# Autodesk Inventor assembly: СборкаЩитков
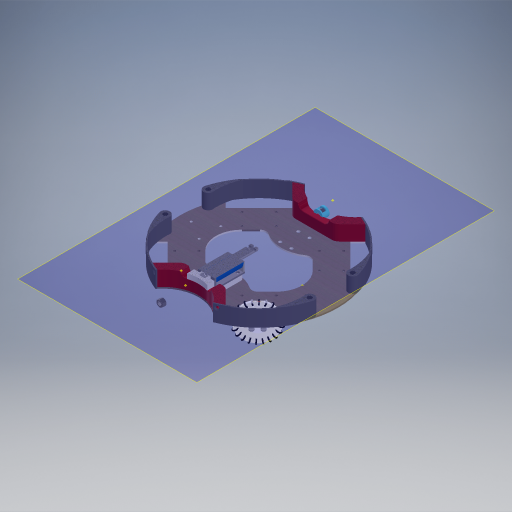
[picture p0: Inventor's stored thumbnail of the model, 512x512]
Saved by Autodesk Inventor 2023 (Build 270158000, 158)
## iProperties
Created: 2025-03-26
Part Number: СборкаЩитков
Document SubType Name: Assembly
Designer: Ivan
Author: Ivan
## Documents named in this file (14)
- C:\!projects\dash_localDirectory\DASH_\Dash-V1\СборкаЩитков.iam
- C:\!projects\dash_localDirectory\DASH_\Dash-V1\step\m3_bolt\СтойкаКруглая.iam
- C:\!projects\dash_localDirectory\DASH_\Dash-V1\floor_v3.ipt
- C:\!projects\dash_localDirectory\DASH_\Dash-V1\contour_v2.ipt
- C:\!projects\dash_localDirectory\DASH_\Dash-V1\protect_v2.2.ipt
- C:\!projects\dash_localDirectory\DASH_\Dash-V1\protect_v2.2_dash.ipt
- C:\!projects\dash_localDirectory\DASH_\Dash-V1\catch_v2.ipt
- C:\!projects\dash_localDirectory\DASH_\Dash-V1\Solenoid\kicker.ipt
- C:\Users\Ivan\Documents\Inventor\Content Center Files\R2023\ru-RU\ANSI B18.2.4.2M\ANSI B18.2.4.2M - M5x0,8 - 8.ipt
- C:\!projects\dash_localDirectory\DASH_\Dash-V1\Solenoid\kicker_MIR.ipt
- C:\!projects\dash_localDirectory\DASH_\Dash-V1\wheel\Wheel.iam
- C:\!projects\DASH-\3D\Dash-V1\Solenoid\Подставка под солноид.ipt
- C:\!projects\DASH-\3D\Dash-V1\Solenoid\Solenoid.iam
- C:\!projects\DASH-\3D\Dash-V1\Solenoid\kicker1.1.ipt
## Components (20 placed, 12 different names)
1. СтойкаКруглая:1 [sub-assembly] — Вставка:19, Вставка:21
2. СтойкаКруглая:2 [sub-assembly] — Вставка:17, Вставка:23
3. СтойкаКруглая:3 [sub-assembly] — Вставка:16, Вставка:22
4. СтойкаКруглая:4 [sub-assembly] — Вставка:18, Вставка:20
5. floor_v3:1 — Вставка:11, Вставка:12, Вставка:13, Касательность:1, Касательность:2, Касательность:3, Касательность:4, Совмещение:6, Совмещение:9, Совмещение:10, Совмещение:11, Вставка:26
6. contour:1 — Вставка:14, Вставка:15, Вставка:16, Вставка:17, Вставка:18, Вставка:19, Угол:2, Совмещение:4, Совмещение:5, Совмещение:7, Совмещение:8
7. protect_v2:1 — Вставка:22, Касательность:1
8. protect_v2:2 — Вставка:20, Касательность:2
9. protect_v2:3 — Вставка:21, Касательность:4
10. protect_v2:4 — Касательность:3, Вставка:23, Совмещение:1, Совмещение:2
11. catch_v2:1 — Вставка:12, Вставка:13, Вставка:15, Совмещение:3
12. catch_v2:2 — Вставка:11, Вставка:14, Совмещение:1, Совмещение:2, Совмещение:13, Заподлицо:2, Совмещение:16
13. kicker:1 — Совмещение:3, Вставка:24, Угол:1, Угол:2
14. ANSI B18.2.4.2M M5x0,8:1 — Вставка:24, Угол:1
15. kicker_MIR:1 — Угол:3, Вставка:25
16. ANSI B18.2.4.2M M5x0,8:2 — Угол:3, Вставка:25
17. Wheel:1 [sub-assembly] — Совмещение:10
18. Подставка под солноид:1 — Совмещение:11, Вставка:26, Совмещение:12, Угол:4, Вставка:27
19. Solenoid:1 [sub-assembly] — Совмещение:12, Угол:4, Вставка:27, Заподлицо:1
20. kicker1.1:1 — Заподлицо:1, Совмещение:13, Заподлицо:2, Совмещение:14, Совмещение:15
## Relationships (43: Insert 17, Mate 16, Tangent 4, Angle 4, Flush 2)
- Вставка:11 [Insert]: floor_v3:1 ↔ catch_v2:2
- Вставка:12 [Insert]: floor_v3:1 ↔ catch_v2:1
- Вставка:13 [Insert]: floor_v3:1 ↔ catch_v2:1
- Вставка:14 [Insert]: contour:1 ↔ catch_v2:2
- Вставка:15 [Insert]: contour:1 ↔ catch_v2:1
- Вставка:16 [Insert]: СтойкаКруглая:3 ↔ contour:1
- Вставка:17 [Insert]: СтойкаКруглая:2 ↔ contour:1
- Вставка:18 [Insert]: СтойкаКруглая:4 ↔ contour:1
- Вставка:19 [Insert]: СтойкаКруглая:1 ↔ contour:1
- Вставка:20 [Insert]: СтойкаКруглая:4 ↔ protect_v2:2
- Вставка:21 [Insert]: СтойкаКруглая:1 ↔ protect_v2:3
- Вставка:22 [Insert]: СтойкаКруглая:3 ↔ protect_v2:1
- Касательность:1 [Tangent]: floor_v3:1 ↔ protect_v2:1
- Касательность:2 [Tangent]: floor_v3:1 ↔ protect_v2:2
- Касательность:3 [Tangent]: floor_v3:1 ↔ protect_v2:4
- Вставка:23 [Insert]: СтойкаКруглая:2 ↔ protect_v2:4
- Касательность:4 [Tangent]: floor_v3:1 ↔ protect_v2:3
- Совмещение:1 [Mate]: protect_v2:4 ↔ catch_v2:2
- Совмещение:2 [Mate]: protect_v2:4 ↔ catch_v2:2
- Совмещение:3 [Mate]: catch_v2:1 ↔ kicker:1
- Вставка:24 [Insert]: kicker:1 ↔ ANSI B18.2.4.2M M5x0,8:1
- Угол:1 [Angle] (0 deg): kicker:1 ↔ ANSI B18.2.4.2M M5x0,8:1
- Угол:2 [Angle] (90 deg): contour:1 ↔ kicker:1
- Совмещение:4 [Mate]: contour:1
- Совмещение:5 [Mate]: contour:1
- Совмещение:6 [Mate]: floor_v3:1
- Совмещение:7 [Mate]: contour:1
- Совмещение:8 [Mate]: contour:1
- Совмещение:9 [Mate]: floor_v3:1
- Угол:3 [Angle] (0 deg): kicker_MIR:1 ↔ ANSI B18.2.4.2M M5x0,8:2
- Вставка:25 [Insert]: kicker_MIR:1 ↔ ANSI B18.2.4.2M M5x0,8:2
- Совмещение:10 [Mate]: floor_v3:1 ↔ Wheel:1
- Совмещение:11 [Mate]: floor_v3:1 ↔ Подставка под солноид:1
- Вставка:26 [Insert]: floor_v3:1 ↔ Подставка под солноид:1
- Совмещение:12 [Mate]: Подставка под солноид:1 ↔ Solenoid:1
- Угол:4 [Angle] (0 deg): Подставка под солноид:1 ↔ Solenoid:1
- Вставка:27 [Insert]: Подставка под солноид:1 ↔ Solenoid:1
- Заподлицо:1 [Flush]: Solenoid:1 ↔ kicker1.1:1
- Совмещение:13 [Mate]: catch_v2:2 ↔ kicker1.1:1
- Заподлицо:2 [Flush]: catch_v2:2 ↔ kicker1.1:1
- Совмещение:14 [Mate]: kicker1.1:1
- Совмещение:15 [Mate]: kicker1.1:1
- Совмещение:16 [Mate]: catch_v2:2
